# Autodesk Inventor assembly: front_right
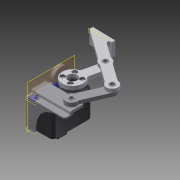
[picture p0: Inventor's stored thumbnail of the model, 180x180]
Saved by Autodesk Inventor 2014 (Build 180170000, 170)
## iProperties
Created: 2015-03-09
Part Number: front_right
Document SubType Name: Assembly
Designer: Hideyuki Takei
Author: Hideyuki Takei
## Documents named in this file (7)
- C:\Users\hide\Desktop\soth-bonsai\cad\front-right.iam
- C:\Users\hide\Desktop\soth-bonsai\cad\RS304MD-ServoHorn.ipt
- C:\Users\hide\Desktop\soth-bonsai\cad\RS304md-simple.ipt
- C:\Users\hide\Desktop\soth-bonsai\cad\servo-holder.ipt
- C:\Users\hide\Desktop\soth-bonsai\cad\link-long.ipt
- C:\Users\hide\Desktop\soth-bonsai\cad\link-short.ipt
- C:\Users\hide\Desktop\soth-bonsai\cad\leg.ipt
## Components (6 placed, 6 different names)
1. RS304MD-ServoHorn:1 — メイト:2, メイト:3, メイト:18
2. RS304md-simple:1 — メイト:2, メイト:3, メイト:5, メイト:6, メイト:10, メイト:25
3. servo-holder:1 — メイト:5, メイト:6, メイト:16, メイト:17, メイト:19, メイト:20, メイト:25
4. link-long:1 — メイト:19, メイト:20, メイト:21, メイト:22
5. link-short:1 — メイト:10, メイト:18, メイト:23
6. leg:1 — メイト:21, メイト:22, メイト:23
## Relationships (14: Mate 14)
- メイト:2 [Mate]: RS304MD-ServoHorn:1 ↔ RS304md-simple:1
- メイト:3 [Mate]: RS304MD-ServoHorn:1 ↔ RS304md-simple:1
- メイト:5 [Mate]: RS304md-simple:1 ↔ servo-holder:1
- メイト:6 [Mate]: RS304md-simple:1 ↔ servo-holder:1
- メイト:10 [Mate]: RS304md-simple:1 ↔ link-short:1
- メイト:16 [Mate]: servo-holder:1
- メイト:17 [Mate]: servo-holder:1
- メイト:18 [Mate]: RS304MD-ServoHorn:1 ↔ link-short:1
- メイト:19 [Mate]: servo-holder:1 ↔ link-long:1
- メイト:20 [Mate]: servo-holder:1 ↔ link-long:1
- メイト:21 [Mate]: link-long:1 ↔ leg:1
- メイト:22 [Mate]: link-long:1 ↔ leg:1
- メイト:23 [Mate]: link-short:1 ↔ leg:1
- メイト:25 [Mate]: RS304md-simple:1 ↔ servo-holder:1
